# Autodesk Inventor assembly: 2020Robot
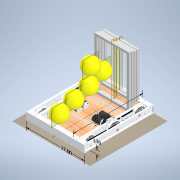
[picture p0: Inventor's stored thumbnail of the model, 180x180]
Saved by Autodesk Inventor 2020.2 (Build 242310000, 310)
## iProperties
Created: 2020-01-09
Part Number: 2020Robot
Document SubType Name: Assembly
Designer: steele
Author: steele
## Documents named in this file (10)
- C:\git\CAD-Development\robSteele\2020LongRobotBase\2020Robot.iam
- C:\git\CAD-Development\robSteele\2020LongRobotBase\AM14U4 Long.iam
- C:\git\CAD-Development\robSteele\2020LongRobotBase\baseForLongRobot.ipt
- C:\git\CAD-Development\robSteele\2020LongRobotBase\1892-YEL.ipt
- C:\git\CAD-Development\robSteele\2020LongRobotBase\floor.ipt
- C:\git\CAD-Development\robSteele\2020LongRobotBase\ceiling.ipt
- C:\git\CAD-Development\robSteele\2020LiftMechanism\primate1stStageForShortRobot.ipt
- C:\git\CAD-Development\robSteele\2020LiftMechanism\primativeBaseForShortRobot.ipt
- C:\git\CAD-Development\robSteele\2020LiftMechanism\primate3rdStageForShortRobot.ipt
- C:\git\CAD-Development\robSteele\2020LiftMechanism\primate4thStageForShortRobot.ipt
## Components (13 placed, 9 different names)
1. AM14U4 Long:1 [sub-assembly] — Mate:1, Mate:2, Mate:3, Mate:6, Mate:19
2. baseForLongRobot:1 — Mate:1, Mate:2, Mate:3, Mate:4, Mate:5, Mate:7, Mate:9, Mate:13, Mate:14, Mate:15, Mate:16, Mate:17, Mate:18, Flush:1
3. 1892-YEL:1 — Mate:13
4. 1892-YEL:2 — Mate:14
5. 1892-YEL:3 — Mate:15
6. 1892-YEL:4 — Mate:16
7. 1892-YEL:5 — Mate:17
8. floor:1 — Mate:4, Mate:5, Mate:6, Mate:8
9. ceiling:1 — Mate:7, Mate:8, Mate:9
10. primativeBaseForShortRobot:1 — Mate:18, Mate:19, Flush:1, Mate:20, Mate:21
11. primate1stStageForShortRobot:1 — Mate:20, Mate:21, Mate:22, Mate:23
12. primate3rdStageForShortRobot:1 — Mate:22, Mate:23, Mate:24, Mate:25
13. primate4thStageForShortRobot:1 — Mate:24, Mate:25
## Relationships (23: Mate 22, Flush 1)
- Mate:1: AM14U4 Long:1 ↔ baseForLongRobot:1
- Mate:2: AM14U4 Long:1 ↔ baseForLongRobot:1
- Mate:3: AM14U4 Long:1 ↔ baseForLongRobot:1
- Mate:4: baseForLongRobot:1 ↔ floor:1
- Mate:5: baseForLongRobot:1 ↔ floor:1
- Mate:6 (48.006 mm): AM14U4 Long:1 ↔ floor:1
- Mate:7: baseForLongRobot:1 ↔ ceiling:1
- Mate:8 (685.8 mm): floor:1 ↔ ceiling:1
- Mate:9: baseForLongRobot:1 ↔ ceiling:1
- Mate:13: baseForLongRobot:1 ↔ 1892-YEL:1
- Mate:14: baseForLongRobot:1 ↔ 1892-YEL:2
- Mate:15: baseForLongRobot:1 ↔ 1892-YEL:3
- Mate:16: baseForLongRobot:1 ↔ 1892-YEL:4
- Mate:17: baseForLongRobot:1 ↔ 1892-YEL:5
- Mate:18: baseForLongRobot:1 ↔ primativeBaseForShortRobot:1
- Mate:19 (76.2 mm): AM14U4 Long:1 ↔ primativeBaseForShortRobot:1
- Flush:1: baseForLongRobot:1 ↔ primativeBaseForShortRobot:1
- Mate:20: primativeBaseForShortRobot:1 ↔ primate1stStageForShortRobot:1
- Mate:21 (6.35 mm): primativeBaseForShortRobot:1 ↔ primate1stStageForShortRobot:1
- Mate:22: primate1stStageForShortRobot:1 ↔ primate3rdStageForShortRobot:1
- Mate:23 (6.35 mm): primate1stStageForShortRobot:1 ↔ primate3rdStageForShortRobot:1
- Mate:24: primate3rdStageForShortRobot:1 ↔ primate4thStageForShortRobot:1
- Mate:25 (6.35 mm): primate3rdStageForShortRobot:1 ↔ primate4thStageForShortRobot:1
